# Autodesk Inventor assembly: Bolt Nut Washer assem
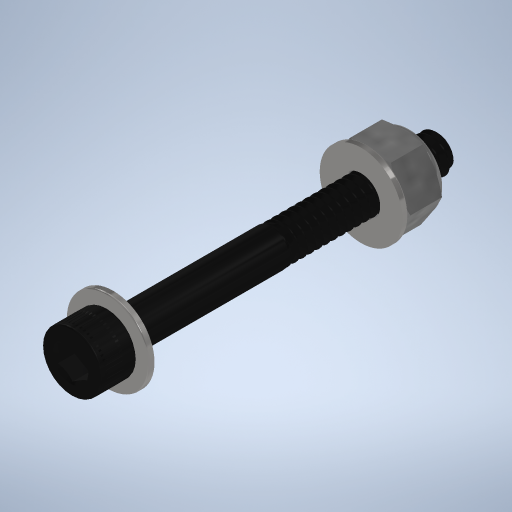
[picture p0: Inventor's stored thumbnail of the model, 512x512]
Saved by Autodesk Inventor 2024 (Build 280153000, 153)
## iProperties
Created: 2023-04-07
Part Number: Bolt Nut Washer assem
Document SubType Name: Assembly
Designer: Dave
Author: Dave
## Documents named in this file (4)
- C:\Users\tangl\OneDrive\Documents\GitHub\BehrendURCMechanical\CAD\Chassis V3\Bolt Nut Washer assem.iam
- C:\Users\tangl\OneDrive\Documents\GitHub\BehrendURCMechanical\CAD\Chassis V3\90107A011_316 Stainless Steel Washer.ipt
- C:\Users\tangl\OneDrive\Documents\GitHub\BehrendURCMechanical\CAD\Chassis V3\91251A252_Black-Oxide Alloy Steel Socket Head Screw.ipt
- C:\Users\tangl\OneDrive\Documents\GitHub\BehrendURCMechanical\CAD\Chassis V3\91831A011_18-8 Stainless Steel Nylon-Insert Locknut.ipt
## Components (4 placed, 3 different names)
1. 90107A011_316 Stainless Steel Washer:1 — Mate:1, Mate:2, Insert:2
2. 91251A252_Black-Oxide Alloy Steel Socket Head Screw:1 — Insert:1, Mate:2
3. 91831A011_18-8 Stainless Steel Nylon-Insert Locknut:1 — Insert:2
4. 90107A011_316 Stainless Steel Washer:2 — Insert:1, Mate:1
## Relationships (4: Insert 2, Mate 2)
- Insert:1: 91251A252_Black-Oxide Alloy Steel Socket Head Screw:1 ↔ 90107A011_316 Stainless Steel Washer:2
- Mate:1 (33.3629 mm): 90107A011_316 Stainless Steel Washer:1 ↔ 90107A011_316 Stainless Steel Washer:2
- Mate:2: 90107A011_316 Stainless Steel Washer:1 ↔ 91251A252_Black-Oxide Alloy Steel Socket Head Screw:1
- Insert:2: 90107A011_316 Stainless Steel Washer:1 ↔ 91831A011_18-8 Stainless Steel Nylon-Insert Locknut:1
